# Autodesk Inventor assembly: fast_akkum
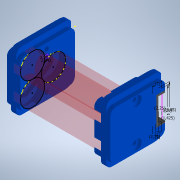
[picture p0: Inventor's stored thumbnail of the model, 180x180]
Saved by Autodesk Inventor 2020 (Build 240168000, 168)
## iProperties
Created: 2022-07-18
Part Number: fast_akkum
Document SubType Name: Assembly
Designer: akapu
Author: akapu
## Documents named in this file (4)
- C:\Users\akapu\Documents\maze bot\fast_akkum.iam
- C:\Users\akapu\Documents\maze bot\fast_battery2.ipt
- C:\Users\akapu\Documents\maze bot\fast_battery.ipt
- C:\Users\akapu\Documents\maze bot\18650.ipt
## Components (3 placed, 3 different names)
1. fast_battery2:1 — Жесткий:1, С поворотом:1
2. fast_battery:1 — Жесткий:1
3. 18650:1 — С поворотом:1
## Relationships (2: WeldJoint 1, RevoluteJoint 1)
- Жесткий:1 [WeldJoint] (3 mm): fast_battery2:1 ↔ fast_battery:1
- С поворотом:1 [RevoluteJoint]: fast_battery2:1 ↔ 18650:1
